# Autodesk Inventor assembly: Assembly
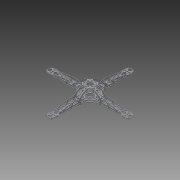
[picture p0: Inventor's stored thumbnail of the model, 180x180]
Saved by Autodesk Inventor 2014 SP1 (Build 180222100, 222)
## iProperties
Created: 2014-07-29
Part Number: Assembly
Document SubType Name: Assembly
Designer: Ryan
Author: Ryan
## Documents named in this file (7)
- C:\Users\Ryan\Documents\Inventor\Quadrocopter\Frame_V1\V1\Assembly.iam
- C:\Users\Ryan\Documents\Inventor\Quadrocopter\Frame_V1\V1\Middle Plate Under.ipt
- C:\Users\Ryan\Documents\Inventor\Quadrocopter\Frame_V1\V1\Arms.iam
- C:\Users\Ryan\Documents\Inventor\Quadrocopter\Frame_V1\V1\Middle Plate Over.ipt
- C:\Users\Ryan\Documents\Inventor\Quadrocopter\Frame_V1\V1\Side_Part.ipt
- C:\Users\Ryan\Documents\Inventor\Quadrocopter\Frame_V1\V1\Plate2.ipt
- C:\Users\Ryan\Documents\Inventor\Quadrocopter\Frame_V1\V1\Plate1.ipt
## Components (16 placed, 6 different names)
1. Middle Plate Under:1 — Mate:1, Mate:2, Mate:3, Mate:4, Mate:5, Mate:6, Mate:7, Mate:8
2. Arms:1 [sub-assembly] — Mate:7, Mate:8, Mate:9, Mate:10, Mate:11
3. Arms:2 [sub-assembly] — Mate:3, Mate:4
4. Arms:3 [sub-assembly] — Mate:5, Mate:6, Mate:21
5. Arms:4 [sub-assembly] — Mate:1, Mate:2
6. Middle Plate Over:1 — Mate:9, Mate:10, Mate:11, Mate:12, Mate:13, Angle:1, Mate:14, Mate:15, Mate:16, Mate:17, Mate:18, Mate:19, Mate:20, Mate:22, Mate:23, Mate:24, Mate:25, Mate:26, Mate:27, Mate:28, Mate:29, Mate:30, Mate:31, Mate:32, Mate:33, Mate:34, Mate:35, Mate:36
7. Side_Part:1 — Mate:12, Mate:13, Angle:1, Mate:14
8. Side_Part:2 — Mate:15, Mate:16, Mate:17, Mate:39
9. Side_Part:3 — Mate:31, Mate:32, Mate:33
10. Side_Part:4 — Mate:34, Mate:35, Mate:36, Mate:42
11. Side_Part:5 — Mate:28, Mate:29, Mate:30
12. Side_Part:6 — Mate:25, Mate:26, Mate:27
13. Side_Part:7 — Mate:22, Mate:23, Mate:24, Mate:40, Mate:41
14. Side_Part:8 — Mate:18, Mate:19, Mate:20, Mate:21, Mate:37, Mate:38
15. Plate2:1 — Mate:37, Mate:38, Mate:39
16. Plate1:1 — Mate:40, Mate:41, Mate:42
## Relationships (43: Mate 42, Angle 1)
- Mate:1: Middle Plate Under:1 ↔ Arms:4
- Mate:2: Middle Plate Under:1 ↔ Arms:4
- Mate:3: Middle Plate Under:1 ↔ Arms:2
- Mate:4: Middle Plate Under:1 ↔ Arms:2
- Mate:5: Middle Plate Under:1 ↔ Arms:3
- Mate:6: Middle Plate Under:1 ↔ Arms:3
- Mate:7: Middle Plate Under:1 ↔ Arms:1
- Mate:8: Middle Plate Under:1 ↔ Arms:1
- Mate:9: Arms:1 ↔ Middle Plate Over:1
- Mate:10: Arms:1 ↔ Middle Plate Over:1
- Mate:11: Arms:1 ↔ Middle Plate Over:1
- Mate:12: Middle Plate Over:1 ↔ Side_Part:1
- Mate:13: Middle Plate Over:1 ↔ Side_Part:1
- Angle:1 (90 deg): Middle Plate Over:1 ↔ Side_Part:1
- Mate:14: Middle Plate Over:1 ↔ Side_Part:1
- Mate:15: Middle Plate Over:1 ↔ Side_Part:2
- Mate:16: Middle Plate Over:1 ↔ Side_Part:2
- Mate:17: Middle Plate Over:1 ↔ Side_Part:2
- Mate:18: Middle Plate Over:1 ↔ Side_Part:8
- Mate:19: Middle Plate Over:1 ↔ Side_Part:8
- Mate:20: Middle Plate Over:1 ↔ Side_Part:8
- Mate:21: Arms:3 ↔ Side_Part:8
- Mate:22: Middle Plate Over:1 ↔ Side_Part:7
- Mate:23: Middle Plate Over:1 ↔ Side_Part:7
- Mate:24: Middle Plate Over:1 ↔ Side_Part:7
- Mate:25: Middle Plate Over:1 ↔ Side_Part:6
- Mate:26: Middle Plate Over:1 ↔ Side_Part:6
- Mate:27: Middle Plate Over:1 ↔ Side_Part:6
- Mate:28: Middle Plate Over:1 ↔ Side_Part:5
- Mate:29: Middle Plate Over:1 ↔ Side_Part:5
- Mate:30: Middle Plate Over:1 ↔ Side_Part:5
- Mate:31: Middle Plate Over:1 ↔ Side_Part:3
- Mate:32: Middle Plate Over:1 ↔ Side_Part:3
- Mate:33: Middle Plate Over:1 ↔ Side_Part:3
- Mate:34: Middle Plate Over:1 ↔ Side_Part:4
- Mate:35: Middle Plate Over:1 ↔ Side_Part:4
- Mate:36: Middle Plate Over:1 ↔ Side_Part:4
- Mate:37: Side_Part:8 ↔ Plate2:1
- Mate:38: Side_Part:8 ↔ Plate2:1
- Mate:39: Side_Part:2 ↔ Plate2:1
- Mate:40: Side_Part:7 ↔ Plate1:1
- Mate:41: Side_Part:7 ↔ Plate1:1
- Mate:42: Side_Part:4 ↔ Plate1:1
